# Autodesk Inventor assembly: FLUGGER TRAY GUIDE ASSY
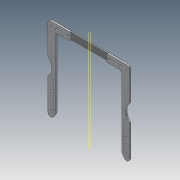
[picture p0: Inventor's stored thumbnail of the model, 180x180]
Saved by Autodesk Inventor 2020.3 (Build 243373000, 373)
## iProperties
RuleStatus: InUse
AfterDocSave0: file://Part Number Cleaner
Created: 2019-10-28
Vendor: HHMI: JRC - ID&F
Document SubType Name: Assembly
Designer: arnoldj
DESIGN DEPARTMENT: HHMI: JRC - ID&F
ALTERED ITEM PART NUMBER: N/A
ALTERED ITEM VENDOR: N/A
ALTERED ITEM DESCRIPTION: N/A
Author: arnoldj
Revision Number: 0
## Documents named in this file (3)
- C:\_WORKSPACE\DATA\PROJECTS\_PROJECTS BY LAB\CARD (LAB)\FLUGGER\FLUGGER TRAY GUIDE ASSY.iam
- C:\_WORKSPACE\DATA\PROJECTS\_PROJECTS BY LAB\FLY FACILITY\FLY MEDIA VIAL PLUGGING\VP TRAY GUIDE SPLIT SHELF.ipt
- C:\_WORKSPACE\DATA\PROJECTS\_PROJECTS BY LAB\FLY FACILITY\FLY MEDIA VIAL PLUGGING\VP TRAY GUIDE CONNECTOR SHELF.ipt
## Components (3 placed, 2 different names)
1. VP TRAY GUIDE SPLIT SHELF:1 — Mate:5, Mate:6, Mate:7
2. VP TRAY GUIDE SPLIT SHELF:2
3. VP TRAY GUIDE CONNECTOR SHELF:1 — Mate:5, Mate:6, Mate:7
## Relationships (3: Mate 3)
- Mate:5: VP TRAY GUIDE SPLIT SHELF:1 ↔ VP TRAY GUIDE CONNECTOR SHELF:1
- Mate:6: VP TRAY GUIDE SPLIT SHELF:1 ↔ VP TRAY GUIDE CONNECTOR SHELF:1
- Mate:7: VP TRAY GUIDE SPLIT SHELF:1 ↔ VP TRAY GUIDE CONNECTOR SHELF:1
